# Autodesk Inventor assembly: TONGKAT ASELOLE
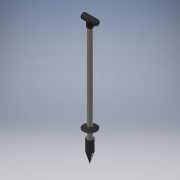
[picture p0: Inventor's stored thumbnail of the model, 180x180]
Saved by Autodesk Inventor 2019.5 (Build 235369000, 369)
## iProperties
Created: 2022-10-11
Part Number: TONGKAT ASELOLE
Document SubType Name: Assembly
Designer: ASUS
Author: ASUS
## Documents named in this file (10)
- C:\Users\ASUS\Downloads\produk fri-074\TONGKAT ASELOLE.iam
- C:\Users\ASUS\Downloads\produk fri-074\penyambung.ipt
- C:\Users\ASUS\Downloads\produk fri-074\badan lampu.ipt
- C:\Users\ASUS\Downloads\produk fri-074\kaca lampu.ipt
- C:\Users\ASUS\Downloads\produk fri-074\ttp lmp.iam
- C:\Users\ASUS\Downloads\produk fri-074\kaca.ipt
- C:\Users\ASUS\Downloads\produk fri-074\Tongkatttt.ipt
- C:\Users\ASUS\Downloads\produk fri-074\Penahan tanah.ipt
- C:\Users\ASUS\Downloads\produk fri-074\ujung tongkat.ipt
- C:\Users\ASUS\Downloads\produk fri-074\termo.ipt
## Components (9 placed, 9 different names)
1. penyambung:2 — Insert:1, Rigid:1, Rotational:2, Mate:3
2. badan lampu:1 — Rotational:1
3. kaca lampu:1 — Rotational:1, Insert:1, Mate:1
4. ttp lmp:1 [sub-assembly] — Rigid:1
5. kaca:2 — Mate:1
6. Tongkatttt:1 — Rotational:2, Rotational:3, Mate:2
7. ujung tongkat:2 — Rotational:3
8. Penahan tanah:2 — Mate:2
9. termo:2 — Mate:3
## Relationships (8: RevoluteJoint 3, Mate 3, Insert 1, WeldJoint 1)
- Rotational:1 [RevoluteJoint]: badan lampu:1 ↔ kaca lampu:1
- Insert:1: penyambung:2 ↔ kaca lampu:1
- Rigid:1 [WeldJoint]: penyambung:2 ↔ ttp lmp:1
- Mate:1: kaca lampu:1 ↔ kaca:2
- Rotational:2 [RevoluteJoint]: penyambung:2 ↔ Tongkatttt:1
- Rotational:3 [RevoluteJoint]: Tongkatttt:1 ↔ ujung tongkat:2
- Mate:2: Tongkatttt:1 ↔ Penahan tanah:2
- Mate:3: penyambung:2 ↔ termo:2
